# Autodesk Inventor assembly: EnsambleW5100
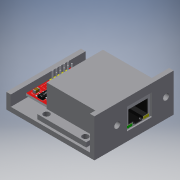
[picture p0: Inventor's stored thumbnail of the model, 180x180]
Saved by Autodesk Inventor 2017 (Build 210142000, 142)
## iProperties
Created: 2021-08-13
Part Number: EnsambleW5100
Document SubType Name: Assembly
Designer: USUARIO
Author: USUARIO
## Documents named in this file (4)
- D:\Laboratorio\Camara Climatica\2021\Camara Climatica Peltier Touch Asemp Zomac SAS 256L #0045886XX OP2021161\Modelo 3D\EnsambleW5100.iam
- D:\Laboratorio\Camara Climatica\2021\Camara Climatica Peltier Touch Asemp Zomac SAS 256L #0045886XX OP2021161\Modelo 3D\W5100_RJ45.ipt
- D:\Laboratorio\Camara Climatica\2021\Camara Climatica Peltier Touch Asemp Zomac SAS 256L #0045886XX OP2021161\Modelo 3D\SoporteEthernet.ipt
- D:\Laboratorio\Camara Climatica\2021\Camara Climatica Peltier Touch Asemp Zomac SAS 256L #0045886XX OP2021161\Modelo 3D\AprieteEthernet.ipt
## Components (3 placed, 3 different names)
1. W5100_RJ45:1 — Mate:1, Flush:1, Mate:2, Mate:3
2. SoporteEthernet:1 — Mate:1, Flush:1, Mate:2, Mate:4
3. AprieteEthernet:1 — Mate:3, Mate:4
## Relationships (5: Mate 4, Flush 1)
- Mate:1: W5100_RJ45:1 ↔ SoporteEthernet:1
- Flush:1 (3 mm): W5100_RJ45:1 ↔ SoporteEthernet:1
- Mate:2 (0.5 mm): W5100_RJ45:1 ↔ SoporteEthernet:1
- Mate:3: W5100_RJ45:1 ↔ AprieteEthernet:1
- Mate:4 (2.5 mm): SoporteEthernet:1 ↔ AprieteEthernet:1
